# Autodesk Inventor assembly: 200-ROCKER-ASM-02
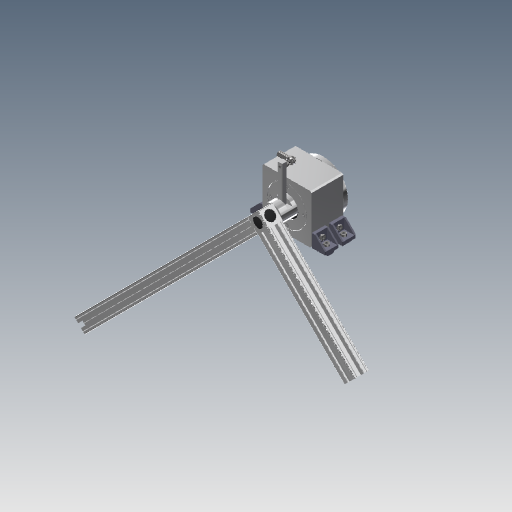
[picture p0: Inventor's stored thumbnail of the model, 512x512]
Saved by Autodesk Inventor 2018.2 (Build 222227000, 227)
## iProperties
Created: 2017-10-30
Part Number: 200-ROCKER-ASM-02
Document SubType Name: Assembly
Designer: Martin Fees
Author: Martin Fees
## Documents named in this file (3)
- D:\Programmierung\FRANC0R\CAD\02-Rocker-Bogie-Robot\200-ROCKER-BOGIE\200-ROCKER-ASM-02.iam
- D:\Programmierung\FRANC0R\CAD\02-Rocker-Bogie-Robot\200-ROCKER-BOGIE\200-10-ROCKER-BEARING\200-10-ROCKER-BEARING-ASM-01.iam
- D:\Programmierung\FRANC0R\CAD\02-Rocker-Bogie-Robot\200-ROCKER-BOGIE\200-20-ROCKER-CONNECTOR\200-20-ROCKER-CONNECTOR-ASM-02.iam
## Components (2 placed, 2 different names)
1. 200-10-ROCKER-BEARING-ASM-01:1 [sub-assembly] — Passend:1, Passend:2, Winkel:1
2. 200-20-ROCKER-CONNECTOR-ASM-02:1 [sub-assembly] — Passend:1, Passend:2, Winkel:1
## Relationships (3: Mate 2, Angle 1)
- Passend:1 [Mate]: 200-10-ROCKER-BEARING-ASM-01:1 ↔ 200-20-ROCKER-CONNECTOR-ASM-02:1
- Passend:2 [Mate]: 200-10-ROCKER-BEARING-ASM-01:1 ↔ 200-20-ROCKER-CONNECTOR-ASM-02:1
- Winkel:1 [Angle] (0 deg): 200-10-ROCKER-BEARING-ASM-01:1 ↔ 200-20-ROCKER-CONNECTOR-ASM-02:1
